# Autodesk Inventor assembly: caster assy
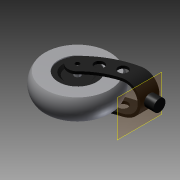
[picture p0: Inventor's stored thumbnail of the model, 180x180]
Saved by Autodesk Inventor 2012 (Build 160160000, 160)
## iProperties
Created: 2012-03-07
Part Number: caster assy
Document SubType Name: Assembly
Designer: esv
Author: esv
## Documents named in this file (3)
- C:\Users\esv\masters\CAD\Invacare\caster assy.iam
- C:\Users\esv\masters\CAD\Invacare\caster wheel.ipt
- C:\Users\esv\masters\CAD\Invacare\caster.ipt
## Components (2 placed, 2 different names)
1. caster wheel:1 — Insert:1
2. caster:1 — Insert:1
## Relationships (1: Insert 1)
- Insert:1: caster wheel:1 ↔ caster:1
